# Autodesk Inventor assembly: ASM_Motor_Unit_Rev_Exploded
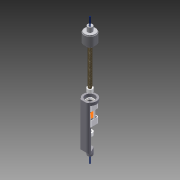
[picture p0: Inventor's stored thumbnail of the model, 180x180]
Saved by Autodesk Inventor 2011 SP2 (Build 150309200, 309)
## iProperties
Created: 2011-09-09
Part Number: ASM_Motor_Unit_Rev_Exploded
Document SubType Name: Assembly
Designer: sungwook
Author: sungwook
## Documents named in this file (4)
- C:\Users\sungwook\Documents\Inventor\Micron20\Assembly\ASM_Motor_Unit_Rev_Exploded.iam
- C:\Users\sungwook\Documents\Inventor\Micron20\Assembly\ASM_Motor_Unit_Part1_Rev.iam
- C:\Users\sungwook\Documents\Inventor\Micron20\Assembly\ASM_Motor_Unit_Part2_Rev.iam
- C:\Users\sungwook\Documents\Inventor\Micron20\Parts\Motor Units\MU_Bottom_Stop.ipt
## Components (3 placed, 3 different names)
1. ASM_Motor_Unit_Part1_Rev:1 [sub-assembly] — Mate:1, Mate:2, Angle:1, Flush:1, Mate:3, Mate:6, Mate:7, Mate:8
2. ASM_Motor_Unit_Part2_Rev:1 [sub-assembly] — Mate:1, Mate:2, Angle:1, Flush:1, Mate:3, Mate:4, Flush:2, Mate:6, Mate:5, Mate:8
3. MU_Bottom_Stop:1 — Mate:4, Flush:2, Mate:5, Mate:7
## Relationships (11: Mate 8, Flush 2, Angle 1)
- Mate:1: ASM_Motor_Unit_Part1_Rev:1 ↔ ASM_Motor_Unit_Part2_Rev:1
- Mate:2: ASM_Motor_Unit_Part1_Rev:1 ↔ ASM_Motor_Unit_Part2_Rev:1
- Angle:1 (180 deg): ASM_Motor_Unit_Part1_Rev:1 ↔ ASM_Motor_Unit_Part2_Rev:1
- Flush:1 (3.4 mm): ASM_Motor_Unit_Part1_Rev:1 ↔ ASM_Motor_Unit_Part2_Rev:1
- Mate:3: ASM_Motor_Unit_Part1_Rev:1 ↔ ASM_Motor_Unit_Part2_Rev:1
- Mate:4: ASM_Motor_Unit_Part2_Rev:1 ↔ MU_Bottom_Stop:1
- Flush:2: ASM_Motor_Unit_Part2_Rev:1 ↔ MU_Bottom_Stop:1
- Mate:5: ASM_Motor_Unit_Part2_Rev:1 ↔ MU_Bottom_Stop:1
- Mate:6 (2.35 mm): ASM_Motor_Unit_Part1_Rev:1 ↔ ASM_Motor_Unit_Part2_Rev:1
- Mate:7: ASM_Motor_Unit_Part1_Rev:1 ↔ MU_Bottom_Stop:1
- Mate:8: ASM_Motor_Unit_Part1_Rev:1 ↔ ASM_Motor_Unit_Part2_Rev:1
